# Autodesk Inventor assembly: Сборка2
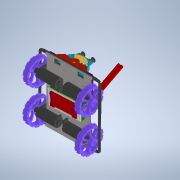
[picture p0: Inventor's stored thumbnail of the model, 180x180]
Saved by Autodesk Inventor 2020 (Build 240168000, 168)
## iProperties
Created: 2022-07-17
Part Number: Сборка2
Document SubType Name: Assembly
Designer: akapu
Author: akapu
## Documents named in this file (22)
- C:\Users\akapu\Documents\maze bot\Сборка2.iam
- C:\Users\akapu\Documents\maze bot\maze_04.ipt
- C:\Users\akapu\Documents\maze bot\motor.ipt
- C:\Users\akapu\Documents\maze bot\motor_ЗЕРКАЛО4.ipt
- C:\Users\akapu\Documents\maze bot\motor_ЗЕРКАЛО_ЗЕРКАЛО.ipt
- C:\Users\akapu\Documents\maze bot\motor_ЗЕРКАЛО5.ipt
- C:\Users\akapu\Documents\maze bot\akkum_holder.ipt
- C:\Users\akapu\Documents\maze bot\metal_holder.ipt
- C:\Users\akapu\Documents\maze bot\fast_akkum2.iam
- C:\Users\akapu\Documents\maze bot\akkum_holder_up.ipt
- C:\Users\akapu\Documents\maze bot\wheel_4.ipt
- C:\Users\akapu\Documents\maze bot\wheel_4_ЗЕРКАЛО.ipt
- C:\Users\akapu\Documents\maze bot\rama.ipt
- C:\Users\akapu\Documents\maze bot\pizza.ipt
- C:\Users\akapu\Documents\maze bot\pizza_disk.ipt
- C:\Users\akapu\Documents\maze bot\pizza_2.ipt
- C:\Users\akapu\Documents\maze bot\vydacha_4.ipt
- C:\Users\akapu\Documents\maze bot\mg996r v17.iam
- C:\Users\akapu\Documents\maze bot\rolik.ipt
- C:\Users\akapu\Documents\maze bot\reyka_3.ipt
- C:\Users\akapu\Documents\maze bot\vagonetka_2.ipt
- C:\Users\akapu\Documents\maze bot\lid.ipt
## Components (24 placed, 21 different names)
1. maze_04:1 — Вставка:1, Совмещение:2, Совмещение:3, Совмещение:4, Совмещение:5, Совмещение:6, Совмещение:7, Совмещение:8, Совмещение:9, Совмещение:11, Вставка:2, С поворотом:10
2. motor:1 — Вставка:1, Совмещение:7, С поворотом:7
3. motor_ЗЕРКАЛО4:1 — Совмещение:3, Совмещение:9, С поворотом:9
4. motor_ЗЕРКАЛО_ЗЕРКАЛО:1 — Совмещение:2, Совмещение:4, Совмещение:8, С поворотом:6
5. motor_ЗЕРКАЛО5:1 — Совмещение:5, Совмещение:6, С поворотом:8
6. fast_akkum2:1 [sub-assembly] — С поворотом:5
7. akkum_holder:1 — Совмещение:11, Совмещение:12
8. metal_holder:1 — Совмещение:12, С поворотом:5
9. akkum_holder_up:1 — Вставка:2
10. wheel_4:3 — С поворотом:6
11. wheel_4:4 — С поворотом:7
12. wheel_4_ЗЕРКАЛО:1 — С поворотом:8
13. wheel_4_ЗЕРКАЛО:2 — С поворотом:9
14. rama:1 — С поворотом:10, Вставка:3, Вставка:5
15. pizza:1 — Вставка:3, С поворотом:11, Вставка:4, С поворотом:13, С поворотом:14, Вставка:6
16. pizza_disk:1 — С поворотом:11
17. pizza_2:1 — Вставка:4
18. vydacha_4:1 — Вставка:5, С поворотом:12
19. mg996r v17:1 [sub-assembly] — С поворотом:12
20. rolik:1 — С поворотом:14
21. rolik:2 — С поворотом:13
22. reyka_3:1 — Вставка:6, Совмещение:13, Совмещение:14
23. vagonetka_2:1
24. lid:1 — Совмещение:13, Совмещение:14
## Relationships (28: Mate 12, RevoluteJoint 10, Insert 6)
- Вставка:1 [Insert]: maze_04:1 ↔ motor:1
- Совмещение:2 [Mate]: maze_04:1 ↔ motor_ЗЕРКАЛО_ЗЕРКАЛО:1
- Совмещение:3 [Mate]: maze_04:1 ↔ motor_ЗЕРКАЛО4:1
- Совмещение:4 [Mate]: maze_04:1 ↔ motor_ЗЕРКАЛО_ЗЕРКАЛО:1
- Совмещение:5 [Mate]: maze_04:1 ↔ motor_ЗЕРКАЛО5:1
- Совмещение:6 [Mate]: maze_04:1 ↔ motor_ЗЕРКАЛО5:1
- Совмещение:7 [Mate]: maze_04:1 ↔ motor:1
- Совмещение:8 [Mate]: maze_04:1 ↔ motor_ЗЕРКАЛО_ЗЕРКАЛО:1
- Совмещение:9 [Mate]: maze_04:1 ↔ motor_ЗЕРКАЛО4:1
- Совмещение:11 [Mate]: maze_04:1 ↔ akkum_holder:1
- Совмещение:12 [Mate]: akkum_holder:1 ↔ metal_holder:1
- С поворотом:5 [RevoluteJoint]: fast_akkum2:1 ↔ metal_holder:1
- Вставка:2 [Insert]: maze_04:1 ↔ akkum_holder_up:1
- С поворотом:6 [RevoluteJoint]: motor_ЗЕРКАЛО_ЗЕРКАЛО:1 ↔ wheel_4:3
- С поворотом:7 [RevoluteJoint]: motor:1 ↔ wheel_4:4
- С поворотом:8 [RevoluteJoint]: motor_ЗЕРКАЛО5:1 ↔ wheel_4_ЗЕРКАЛО:1
- С поворотом:9 [RevoluteJoint]: motor_ЗЕРКАЛО4:1 ↔ wheel_4_ЗЕРКАЛО:2
- С поворотом:10 [RevoluteJoint]: maze_04:1 ↔ rama:1
- Вставка:3 [Insert]: rama:1 ↔ pizza:1
- С поворотом:11 [RevoluteJoint]: pizza:1 ↔ pizza_disk:1
- Вставка:4 [Insert]: pizza:1 ↔ pizza_2:1
- Вставка:5 [Insert]: rama:1 ↔ vydacha_4:1
- С поворотом:12 [RevoluteJoint]: vydacha_4:1 ↔ mg996r v17:1
- С поворотом:13 [RevoluteJoint]: pizza:1 ↔ rolik:2
- С поворотом:14 [RevoluteJoint]: pizza:1 ↔ rolik:1
- Вставка:6 [Insert]: pizza:1 ↔ reyka_3:1
- Совмещение:13 [Mate]: reyka_3:1 ↔ lid:1
- Совмещение:14 [Mate]: reyka_3:1 ↔ lid:1
